# Autodesk Inventor assembly: GriperBaseV1_2
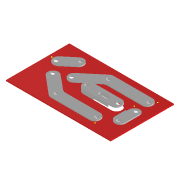
[picture p0: Inventor's stored thumbnail of the model, 180x180]
Saved by Autodesk Inventor 2021 (Build 250183000, 183)
## iProperties
Created: 2022-10-24
Part Number: GriperBaseV1_2
Document SubType Name: Assembly
Designer: brian
Author: brian
## Documents named in this file (2)
- G:\Mi unidad\Universidad\Control\Robotica\Laboratorio\Proyecto\Archivos SAT\GripperBasePick.iam
- G:\Mi unidad\Universidad\Control\Robotica\Laboratorio\Proyecto\GripperBase.iam
## Components (1 placed, 1 different names)
1. GripperBase:1 [sub-assembly] — Flush:2, Mate:2, Mate:3
## Relationships (3: Mate 2, Flush 1)
- Flush:2: GripperBase:1
- Mate:2: GripperBase:1
- Mate:3: GripperBase:1
